# Autodesk Inventor assembly: tracks_test
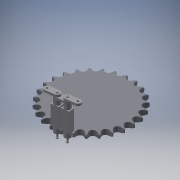
[picture p0: Inventor's stored thumbnail of the model, 180x180]
Saved by Autodesk Inventor 2016 (Build 200138000, 138)
## iProperties
Created: 2016-11-10
Part Number: tracks_test
Document SubType Name: Assembly
Designer: hesaon
Author: hesaon
## Documents named in this file (5)
- D:\documents\SOD-II\cad\tracks_test.iam
- D:\documents\SOD-II\cad\tracks_outer.ipt
- D:\documents\SOD-II\cad\tracks_center_sod_ii.ipt
- D:\documents\SOD-II\cad\screw_Ka22x16.ipt
- D:\documents\SOD-II\cad\dummy_drive_train\Design Accelerator\Roller Chain Sprocket11.ipt
## Components (13 placed, 4 different names)
1. tracks_outer:1 — Insert:6, Flush:5, Insert:10
2. tracks_outer:2 — Insert:1, Insert:2, Flush:1, Insert:7, Insert:8, Flush:2, Flush:3
3. tracks_outer:3 — Insert:5, Flush:4, Insert:9
4. tracks_outer:4 — Insert:3, Insert:4, Insert:5, Insert:6, Flush:4, Flush:5, Mate:1
5. tracks_center_sod_ii:1 — Insert:1, Insert:3, Flush:6
6. tracks_center_sod_ii:2 — Insert:2, Flush:1, Insert:4, Flush:6
7. tracks_outer:5 — Insert:7, Flush:3, Insert:12
8. tracks_outer:6 — Insert:8, Flush:2, Insert:11
9. screw_Ka22x16:1 — Insert:9
10. screw_Ka22x16:2 — Insert:11
11. screw_Ka22x16:3 — Insert:10
12. screw_Ka22x16:4 — Insert:12
13. Roller Chain Sprocket1:1 — Mate:1
## Relationships (19: Insert 12, Flush 6, Mate 1)
- Insert:1: tracks_outer:2 ↔ tracks_center_sod_ii:1
- Insert:2: tracks_outer:2 ↔ tracks_center_sod_ii:2
- Flush:1: tracks_outer:2 ↔ tracks_center_sod_ii:2
- Insert:3: tracks_outer:4 ↔ tracks_center_sod_ii:1
- Insert:4: tracks_outer:4 ↔ tracks_center_sod_ii:2
- Insert:5: tracks_outer:3 ↔ tracks_outer:4
- Insert:6: tracks_outer:1 ↔ tracks_outer:4
- Insert:7: tracks_outer:2 ↔ tracks_outer:5
- Insert:8: tracks_outer:2 ↔ tracks_outer:6
- Flush:2: tracks_outer:2 ↔ tracks_outer:6
- Flush:3: tracks_outer:2 ↔ tracks_outer:5
- Flush:4: tracks_outer:3 ↔ tracks_outer:4
- Flush:5: tracks_outer:1 ↔ tracks_outer:4
- Insert:9: tracks_outer:3 ↔ screw_Ka22x16:1
- Insert:10: tracks_outer:1 ↔ screw_Ka22x16:3
- Insert:11: tracks_outer:6 ↔ screw_Ka22x16:2
- Insert:12: tracks_outer:5 ↔ screw_Ka22x16:4
- Mate:1: tracks_outer:4 ↔ Roller Chain Sprocket1:1
- Flush:6: tracks_center_sod_ii:1 ↔ tracks_center_sod_ii:2
